# Autodesk Inventor assembly: assembly roket
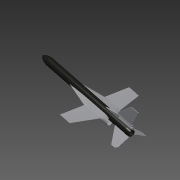
[picture p0: Inventor's stored thumbnail of the model, 180x180]
Saved by Autodesk Inventor 2014 SP1 (Build 180222100, 222)
## iProperties
Created: 2018-05-06
Part Number: assembly roket
Document SubType Name: Assembly
Designer: Dadang
Author: Dadang
## Documents named in this file (6)
- D:\Gambar Inventor\Wahana Roket\assembly roket.iam
- D:\Gambar Inventor\Wahana Roket\Fuselage.ipt
- D:\Gambar Inventor\Wahana Roket\stabillizer.ipt
- D:\Gambar Inventor\Wahana Roket\vertikal stab.ipt
- D:\Gambar Inventor\Wahana Roket\EDF Cone.ipt
- D:\Gambar Inventor\Wahana Roket\wing 2.ipt
## Components (7 placed, 5 different names)
1. Fuselage:1 — Mate:22, Mate:23, Mate:24, Mate:25, Mate:26, Mate:27, Mate:28, Mate:29, Mate:30, Mate:31, Mate:32, Mate:33, Mate:34, Mate:35, Mate:36, Mate:37, Mate:38, Mate:39
2. vertikal stab:1 — Mate:25, Mate:26, Mate:27
3. vertikal stab:2 — Mate:22, Mate:23, Mate:24
4. wing 2:1 — Mate:28, Mate:29, Mate:30
5. wing 2:2 — Mate:31, Mate:32, Mate:33
6. EDF Cone:1 — Mate:34, Mate:35, Mate:36
7. stabillizer:1 — Mate:37, Mate:38, Mate:39
## Relationships (18: Mate 18)
- Mate:22: Fuselage:1 ↔ vertikal stab:2
- Mate:23: Fuselage:1 ↔ vertikal stab:2
- Mate:24: Fuselage:1 ↔ vertikal stab:2
- Mate:25: Fuselage:1 ↔ vertikal stab:1
- Mate:26: Fuselage:1 ↔ vertikal stab:1
- Mate:27: Fuselage:1 ↔ vertikal stab:1
- Mate:28: Fuselage:1 ↔ wing 2:1
- Mate:29: Fuselage:1 ↔ wing 2:1
- Mate:30: Fuselage:1 ↔ wing 2:1
- Mate:31: Fuselage:1 ↔ wing 2:2
- Mate:32: Fuselage:1 ↔ wing 2:2
- Mate:33: Fuselage:1 ↔ wing 2:2
- Mate:34: Fuselage:1 ↔ EDF Cone:1
- Mate:35: Fuselage:1 ↔ EDF Cone:1
- Mate:36: Fuselage:1 ↔ EDF Cone:1
- Mate:37: Fuselage:1 ↔ stabillizer:1
- Mate:38: Fuselage:1 ↔ stabillizer:1
- Mate:39: Fuselage:1 ↔ stabillizer:1
